# Autodesk Inventor assembly: RAMPS Mount
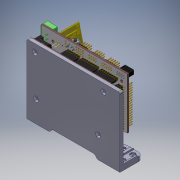
[picture p0: Inventor's stored thumbnail of the model, 180x180]
Saved by Autodesk Inventor 2018 (Build 220112000, 112)
## iProperties
Created: 2018-05-30
Part Number: RAMPS Mount
Document SubType Name: Assembly
Designer: Jasper
Author: Jasper
## Documents named in this file (3)
- C:\Users\Jasper\Downloads\git_WSL\MEME_MACHINE\CAD\RAMPS Mount\RAMPS Mount.iam
- C:\Users\Jasper\Downloads\git_WSL\MEME_MACHINE\CAD\Vitamins\Arduino RAMPS combo.iam
- C:\Users\Jasper\Downloads\git_WSL\MEME_MACHINE\CAD\RAMPS Mount\Mount.ipt
## Components (2 placed, 2 different names)
1. Arduino RAMPS combo:1 [sub-assembly] — Mate:1, Mate:2, Angle:1
2. Mount:1 — Mate:1, Mate:2, Angle:1
## Relationships (3: Mate 2, Angle 1)
- Mate:1: Arduino RAMPS combo:1 ↔ Mount:1
- Mate:2: Arduino RAMPS combo:1 ↔ Mount:1
- Angle:1 (0 deg): Arduino RAMPS combo:1 ↔ Mount:1
